# Autodesk Inventor assembly: FO_020_25_2_03
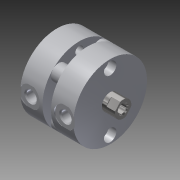
[picture p0: Inventor's stored thumbnail of the model, 180x180]
Saved by Autodesk Inventor 2013 (Build 170138000, 138)
## iProperties
Created: 2013-06-07
Part Number: FO_020_25_2_03
Document SubType Name: Assembly
Designer: mvarma
Author: mvarma
## Documents named in this file (7)
- C:\Users\mvarma\Desktop\GRT 2013-2014 Gearbox\Mark 2\Imported Components\FO_020_25_2_03\FO_020_25_2_03.iam
- C:\Users\mvarma\Desktop\GRT 2013-2014 Gearbox\Mark 2\Imported Components\FO_020_25_2_03\1.ipt
- C:\Users\mvarma\Desktop\GRT 2013-2014 Gearbox\Mark 2\Imported Components\FO_020_25_2_03\2.ipt
- C:\Users\mvarma\Desktop\GRT 2013-2014 Gearbox\Mark 2\Imported Components\FO_020_25_2_03\3.ipt
- C:\Users\mvarma\Desktop\GRT 2013-2014 Gearbox\Mark 2\Imported Components\FO_020_25_2_03\4.ipt
- C:\Users\mvarma\Desktop\GRT 2013-2014 Gearbox\Mark 2\Imported Components\FO_020_25_2_03\5.ipt
- C:\Users\mvarma\Desktop\GRT 2013-2014 Gearbox\Mark 2\Imported Components\FO_020_25_2_03\6.ipt
## Components (9 placed, 6 different names)
1. 1:1 — Mate:3, Mate:4, Mate:25
2. 2:1 — Mate:12, Flush:2, Mate:15, Mate:16
3. 3:1 — Mate:14, Mate:15, Mate:16, Mate:17, Mate:18, Mate:19, Mate:20, Mate:21, Mate:22, Mate:23, Mate:24
4. 4:1 — Mate:13, Flush:1, Mate:14
5. 5:1 — Mate:12, Mate:13, Flush:1, Flush:2
6. 6:1 — Mate:3, Mate:4, Mate:22, Mate:23
7. 6:2 — Mate:17, Mate:18
8. 6:3 — Mate:19, Mate:20, Mate:25
9. 6:4 — Mate:21, Mate:24
## Relationships (18: Mate 16, Flush 2)
- Mate:3: 1:1 ↔ 6:1
- Mate:4: 1:1 ↔ 6:1
- Mate:12: 2:1 ↔ 5:1
- Mate:13: 4:1 ↔ 5:1
- Flush:1: 4:1 ↔ 5:1
- Mate:14: 3:1 ↔ 4:1
- Flush:2: 2:1 ↔ 5:1
- Mate:15: 2:1 ↔ 3:1
- Mate:16: 2:1 ↔ 3:1
- Mate:17: 3:1 ↔ 6:2
- Mate:18: 3:1 ↔ 6:2
- Mate:19: 3:1 ↔ 6:3
- Mate:20: 3:1 ↔ 6:3
- Mate:21: 3:1 ↔ 6:4
- Mate:22: 3:1 ↔ 6:1
- Mate:23: 3:1 ↔ 6:1
- Mate:24: 3:1 ↔ 6:4
- Mate:25: 1:1 ↔ 6:3
